# Autodesk Inventor assembly: stackLight
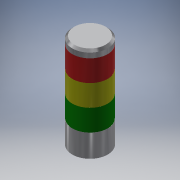
[picture p0: Inventor's stored thumbnail of the model, 180x180]
Saved by Autodesk Inventor 2018 (Build 220112000, 112)
## iProperties
Created: 2017-04-10
Part Number: stackLight
Document SubType Name: Assembly
Designer: dkt01
Author: dkt01
## Documents named in this file (4)
- C:\Users\dktur\Dropbox\StackLightMonitor\CAD\stackLight.iam
- C:\Users\dktur\Dropbox\StackLightMonitor\CAD\stackLightBase.ipt
- C:\Users\dktur\Dropbox\StackLightMonitor\CAD\stackLightElement.ipt
- C:\Users\dktur\Dropbox\StackLightMonitor\CAD\stackLightTop.ipt
## Components (5 placed, 3 different names)
1. stackLightBase:1 — Insert:1
2. stackLightElement:1 — Insert:2, Insert:3
3. stackLightElement:2 — Insert:3, Insert:4
4. stackLightElement:3 — Insert:1, Insert:2
5. stackLightTop:1 — Insert:4
## Relationships (4: Insert 4)
- Insert:1: stackLightBase:1 ↔ stackLightElement:3
- Insert:2: stackLightElement:1 ↔ stackLightElement:3
- Insert:3: stackLightElement:1 ↔ stackLightElement:2
- Insert:4: stackLightElement:2 ↔ stackLightTop:1
